# Autodesk Inventor assembly: Ellbow n24_v2
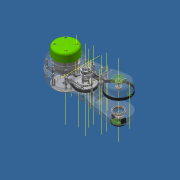
[picture p0: Inventor's stored thumbnail of the model, 180x180]
Saved by Autodesk Inventor 2016 (Build 200138000, 138)
## iProperties
Created: 2015-08-24
Part Number: Ellbow n24_v2
Material: Generisch
Document SubType Name: Assembly
Designer: 4ndreas
Mass: 4151.42 g
Surface Area: 5104.54 cm^2
Volume: 2390.65 cm^3
Density: 1.73652 g/cm^3
Author: 4ndreas
## Documents named in this file (32)
- C:\Users\4ndreas\Documents\Inventor\RobotARM v2\v4\Ellbow n24_v2.iam
- C:\Users\4ndreas\Documents\Inventor\RobotARM v2\v4\Ellbow\Konstruktions-Assistent\Übertragung des Zahnriemens1.iam
- C:\Users\4ndreas\Documents\Inventor\RobotARM v2\v4\Nema24.ipt
- C:\Users\4ndreas\Documents\Inventor\RobotARM v2\v4\Ellbow\Konstruktions-Assistent\Übertragung des Zahnriemens2.iam
- C:\Users\4ndreas\Documents\Inventor\RobotARM v2\v4\OberArm_A.ipt
- C:\Users\4ndreas\Documents\Inventor\RobotARM v2\v4\OberArm_B.ipt
- C:\Users\4ndreas\Documents\Inventor\RobotARM v2\v4\OberArm_C.ipt
- C:\Users\4ndreas\Documents\Inventor\RobotARM v2\v4\Ellbow n24_v2\Konstruktions-Assistent\Welle1.iam
- C:\Users\4ndreas\Documents\Inventor\Content Center Files\R2014\de-DE\DIN BEARING(1)\DIN 625 SKF - SKF 608.ipt
- C:\Users\4ndreas\Documents\Inventor\RobotARM v2\v2\encoder.iam
- C:\Users\4ndreas\Documents\Inventor\RobotARM v2\v4\DIN 912 - M4 x 0,7.ipt
- C:\Users\4ndreas\Documents\Inventor\RobotARM v2\v4\MotorCoverN24_3.ipt
- C:\Users\4ndreas\Documents\Inventor\RobotARM v2\v4\Cover_G2.ipt
- C:\Users\4ndreas\Documents\Inventor\Content Center Files\R2014\de-DE\DIN 912\DIN 912 - M3 x 0,5 x 10 x 8,75.ipt
- C:\Users\4ndreas\Documents\Inventor\Content Center Files\R2014\de-DE\DIN 912\DIN 912 - M4 x 0,7 x 35 x 20.ipt
- C:\Users\4ndreas\Documents\Inventor\Content Center Files\R2014\de-DE\DIN 912\DIN 912 - M4 x 0,7 x 40 x 20.ipt
- C:\Users\4ndreas\Documents\Inventor\Content Center Files\R2014\de-DE\DIN 9021\DIN 9021 - 4,3.ipt
- C:\Users\4ndreas\Documents\Inventor\Content Center Files\R2014\de-DE\DIN 625 - T1\DIN 625 T1 - 624 - 4 x 13 x 5.ipt
- C:\Users\4ndreas\Documents\Inventor\Content Center Files\R2014\de-DE\DIN 125-1  A\DIN 125 - A 4,3.ipt
- C:\Users\4ndreas\Documents\Inventor\RobotARM v2\Diszanzbolzen_M4x20.ipt
- C:\Users\4ndreas\Documents\Inventor\Content Center Files\R2014\de-DE\DIN BEARING(1)\DIN 625 SKF - SKF 61807.ipt
- C:\Users\4ndreas\Documents\Inventor\RobotARM v2\v4\DIN 912 - M4 x 0,7 x55.ipt
- C:\Users\4ndreas\Documents\Inventor\RobotARM v2\v4\16221600.ipt
- C:\Users\4ndreas\Documents\Inventor\RobotARM v2\v4\16224800.ipt
- C:\Users\4ndreas\Documents\Inventor\Content Center Files\R2014\de-DE\DIN 912\DIN 912 - M4 x 0,7 x 30 x 20.ipt
- C:\Users\4ndreas\Documents\Inventor\Content Center Files\R2014\de-DE\DIN 933\DIN 933 - M4  x 55.ipt
- C:\Users\4ndreas\Documents\Inventor\Content Center Files\R2014\de-DE\DIN 934\DIN 934 - M4 x 0,7.ipt
- C:\Users\4ndreas\Documents\Inventor\Content Center Files\R2014\de-DE\DIN 562\DIN 562 - M4 x 7.ipt
- C:\Users\4ndreas\Documents\Inventor\Content Center Files\R2014\de-DE\DIN 933\DIN 933 - M4  x 25.ipt
- C:\Users\4ndreas\Documents\Inventor\RobotARM v2\v4\OberArmMagnet.ipt
- C:\Users\4ndreas\Documents\Inventor\Content Center Files\R2014\de-DE\DIN 7991(2)\DIN 7991 - M4x30.ipt
- C:\Users\4ndreas\Documents\Inventor\Content Center Files\R2014\de-DE\DIN 985\DIN 985 - M4.ipt
## Components (142 placed, 30 different names)
1. Übertragung des Zahnriemens:1 [sub-assembly] — Passend:25, Passend:31, Passend:37, Passend:41, Passend:104, Passend:105, Passend:120, Passend:193
2. Nema24:1 — Passend:3, Passend:16, Winkel:1, Winkel:2, Passend:33, Passend:35, Passend:36, Passend:52, Passend:54, Passend:55, Passend:154, Passend:155, Fluchtend:11
3. Übertragung des Zahnriemens:2 [sub-assembly] — Passend:16, Passend:24, Passend:34, Passend:156
4. OberArm_A:1 — Passend:29, Fluchtend:1, Passend:30, Fluchtend:3, Passend:32, Passend:33, Passend:34, Passend:44, Passend:45, Passend:72, Passend:73, Passend:74, Passend:75, Passend:76, Passend:78, Passend:245, Passend:246, Passend:247, Passend:248, Passend:249
5. OberArm_B:1 — Passend:28, Passend:29, Fluchtend:1, Passend:30, Fluchtend:4, Passend:43, Passend:50, Passend:226, Passend:227, Passend:228, Passend:229, Passend:241, Passend:242, Passend:243, Passend:244, Fluchtend:12
6. OberArm_C:1 — Passend:28, Fluchtend:3, Passend:31, Fluchtend:4, Passend:48, Passend:49, Passend:51, Fluchtend:9, Passend:100, Passend:101, Passend:102, Passend:103, Passend:107, Passend:108, Passend:130, Passend:131, Passend:132, Passend:133, Passend:134, Passend:135, Passend:136, Passend:137, Passend:138, Passend:144, Passend:150, Passend:151, Passend:161, Passend:162, Passend:201, Passend:202, Passend:203, Passend:204, Passend:205, Passend:211, Passend:220, Passend:222, Passend:223, Passend:250, Passend:251, Passend:252, Passend:256
7. Cover_G2:1 — Fluchtend:9, Passend:80, Passend:81, Passend:82, Passend:83, Passend:84, Passend:85, Passend:86, Passend:87
8. Welle:1 [sub-assembly] — Passend:37, Passend:38, Passend:40, Passend:39, Passend:206
9. encoder:1 [sub-assembly] — Passend:41, Passend:43, Passend:256
10. OberArmMagnet:1 — Fluchtend:12, Passend:261, Passend:262, Fluchtend:13, Passend:263, Passend:264, Fluchtend:14, Fluchtend:15
11. DIN 625 SKF SKF 608:1 — Passend:38, Passend:204
12. DIN 625 SKF SKF 608:2 — Passend:39, Passend:205, Passend:207
13. DIN 625 SKF SKF 608:3 — Passend:40, Passend:203
14. DIN 625 SKF SKF 608:4 — Passend:45, Passend:49
15. DIN 625 SKF SKF 608:5 — Passend:50, Passend:51
16. DIN 625 SKF SKF 608:6 — Passend:44, Passend:48
17. DIN 912 - ersetzt durch DIN EN ISO 4762 M4 x 50:5 — Passend:55, Passend:71, Passend:258
18. DIN 912 - ersetzt durch DIN EN ISO 4762 M4 x 50:6 — Passend:54, Passend:69
19. DIN 912 - ersetzt durch DIN EN ISO 4762 M4 x 50:7 — Passend:53, Passend:70
20. DIN 912 - ersetzt durch DIN EN ISO 4762 M4 x 50:8 — Passend:52, Passend:68
21. DIN 125-1 A A 4,3:6
22. DIN 125-1 A A 4,3:7
23. DIN 125-1 A A 4,3:8
24. DIN 125-1 A A 4,3:9
25. Diszanzbolzen_M4x20:5 — Passend:71, Fluchtend:6, Fluchtend:7, Passend:72
26. Diszanzbolzen_M4x20:6 — Passend:69, Fluchtend:6, Passend:73, Passend:88
27. Diszanzbolzen_M4x20:7 — Passend:70, Fluchtend:7, Fluchtend:8, Passend:75, Passend:76
28. Diszanzbolzen_M4x20:8 — Passend:68, Fluchtend:8, Passend:74, Passend:259
29. MotorCoverN24_3:1 — Passend:78, Passend:89, Passend:92, Passend:93, Passend:94, Passend:257, Passend:260
30. DIN 912 - ersetzt durch DIN EN ISO 4762 M3 x 10:1 — Passend:82, Passend:87
31. DIN 912 - ersetzt durch DIN EN ISO 4762 M3 x 10:2 — Passend:81, Passend:86
32. DIN 912 - ersetzt durch DIN EN ISO 4762 M3 x 10:3 — Passend:83, Passend:84
33. DIN 912 - ersetzt durch DIN EN ISO 4762 M3 x 10:4 — Passend:80, Passend:85
34. DIN 912 - ersetzt durch DIN EN ISO 4762 M4 x 35:1 — Passend:88, Passend:89
35. DIN 912 - ersetzt durch DIN EN ISO 4762 M4 x 35:2 — Passend:92, Passend:93, Passend:258
36. DIN 912 - ersetzt durch DIN EN ISO 4762 M4 x 35:3 — Passend:259, Passend:260
37. DIN 912 - ersetzt durch DIN EN ISO 4762 M4 x 35:4 — Passend:90, Passend:94, Passend:257
38. DIN 912 - ersetzt durch DIN EN ISO 4762 M4 x 40:10 — Passend:96, Passend:99, Passend:101, Passend:105, Passend:109, Passend:115, Passend:121, Passend:127
39. DIN 912 - ersetzt durch DIN EN ISO 4762 M4 x 40:9 — Passend:97, Passend:98, Passend:100, Passend:104, Passend:106, Passend:114, Passend:126
40. DIN 9021 4,3:1 — Passend:96, Passend:99, Passend:102
41. DIN 9021 4,3:2 — Passend:97, Passend:98, Passend:103
42. DIN 9021 4,3:3 — Passend:108, Passend:109, Passend:122
43. DIN 9021 4,3:4 — Passend:106, Passend:107, Passend:123
44. DIN 625 - T1 624 - 4 x 13 x 5:1 — Passend:110, Passend:112, Passend:124
45. DIN 625 - T1 624 - 4 x 13 x 5:2 — Passend:110, Passend:112, Passend:115, Passend:129
46. DIN 625 - T1 624 - 4 x 13 x 5:3 — Passend:111, Passend:113, Passend:125
47. DIN 625 - T1 624 - 4 x 13 x 5:4 — Passend:111, Passend:113, Passend:114, Passend:128
48. DIN 125-1 A A 4,3:1 — Passend:117, Passend:119, Passend:125
49. DIN 125-1 A A 4,3:2 — Passend:117, Passend:119, Passend:120, Passend:123
50. DIN 125-1 A A 4,3:3 — Passend:116, Passend:118, Passend:124
51. DIN 125-1 A A 4,3:4 — Passend:116, Passend:118, Passend:121, Passend:122
52. DIN 985 - ersetzt durch DIN EN ISO 10511 M4:1 — Passend:126, Passend:128
53. DIN 985 - ersetzt durch DIN EN ISO 10511 M4:2 — Passend:127, Passend:129
54. DIN 625 SKF SKF 61807:1 — Passend:130, Passend:131
55. Diszanzbolzen_M4x20:9 — Passend:132, Passend:136, Passend:137
56. Diszanzbolzen_M4x20:10 — Passend:133, Passend:134, Passend:135
57. DIN 912 - ersetzt durch DIN EN ISO 4762 M4 x 55:12 — Passend:138
58. DIN 125-1 A A 4,3:10
59. DIN 912 - ersetzt durch DIN EN ISO 4762 M4 x 55:13 — Passend:144
60. DIN 125-1 A A 4,3:11
61. DIN 912 - ersetzt durch DIN EN ISO 4762 M4 x 55:14 — Passend:151
62. DIN 125-1 A A 4,3:12
63. DIN 912 - ersetzt durch DIN EN ISO 4762 M4 x 55:15 — Passend:150
64. DIN 125-1 A A 4,3:13
65. 16221600:1 — Passend:154, Passend:155, Fluchtend:10
66. 16224800:1 — Passend:156, Fluchtend:10
67. DIN 912 - ersetzt durch DIN EN ISO 4762 M4 x 55:16 — Passend:162, Passend:190
68. DIN 912 - ersetzt durch DIN EN ISO 4762 M4 x 55:17 — Passend:161, Passend:165, Passend:188
69. DIN 125-1 A A 4,3:14
70. DIN 125-1 A A 4,3:15
71. DIN 912 - ersetzt durch DIN EN ISO 4762 M4 x 30:1 — Passend:165, Passend:187
72. DIN 125-1 A A 4,3:16
73. DIN 125-1 A A 4,3:17
74. DIN 933 - ersetzt durch DIN EN 24017 M4  x 55:2 — Passend:184, Passend:191, Passend:192, Passend:198
75. DIN 933 - ersetzt durch DIN EN 24017 M4  x 55:1 — Passend:183, Passend:194, Passend:196
76. DIN 125-1 A A 4,3:18
77. DIN 125-1 A A 4,3:19
78. DIN 934 - ersetzt durch DIN EN 24032/28673/28674 M4:1 — Passend:188
79. DIN 934 - ersetzt durch DIN EN 24032/28673/28674 M4:2 — Passend:187
80. DIN 934 - ersetzt durch DIN EN 24032/28673/28674 M4:3 — Passend:184
81. DIN 934 - ersetzt durch DIN EN 24032/28673/28674 M4:4 — Passend:183
82. DIN 934 - ersetzt durch DIN EN 24032/28673/28674 M4:6 — Passend:190
83. DIN 625 - T1 624 - 4 x 13 x 5:5 — Passend:193, Passend:195, Passend:197
84. DIN 625 - T1 624 - 4 x 13 x 5:6 — Passend:192, Passend:199, Passend:201
85. DIN 625 - T1 624 - 4 x 13 x 5:7 — Passend:191, Passend:199, Passend:200
86. DIN 625 - T1 624 - 4 x 13 x 5:8 — Passend:194, Passend:195, Passend:202
87. DIN 934 - ersetzt durch DIN EN 24032/28673/28674 M4:7 — Passend:196, Passend:197
88. DIN 934 - ersetzt durch DIN EN 24032/28673/28674 M4:8 — Passend:198, Passend:200
89. 16221600:2 — Passend:206, Passend:207
90. DIN 912 - ersetzt durch DIN EN ISO 4762 M4 x 55:18 — Passend:211, Passend:239
91. DIN 125-1 A A 4,3:20
92. DIN 912 - ersetzt durch DIN EN ISO 4762 M4 x 55:19 — Passend:220, Passend:240
93. DIN 912 - ersetzt durch DIN EN ISO 4762 M4 x 55:20 — Passend:222, Passend:238
94. DIN 912 - ersetzt durch DIN EN ISO 4762 M4 x 55:21 — Passend:223, Passend:237
95. DIN 125-1 A A 4,3:21
96. DIN 125-1 A A 4,3:5
97. DIN 125-1 A A 4,3:22
98. DIN 562 M4:1 — Passend:239, Passend:245, Passend:246
99. DIN 562 M4:2 — Passend:240, Passend:241, Passend:242
100. DIN 562 M4:3 — Passend:237, Passend:247, Passend:248
101. DIN 562 M4:4 — Passend:238, Passend:243, Passend:244
102. DIN 933 - ersetzt durch DIN EN 24017 M4  x 25:1 — Passend:250, Passend:251, Passend:252, Passend:254
103. DIN 934 - ersetzt durch DIN EN 24032/28673/28674 M4:9 — Passend:254
104. DIN 7991 M4x30:2 — Passend:262, Fluchtend:13
105. DIN 7991 M4x30:3 — Passend:263, Fluchtend:14
106. DIN 7991 M4x30:4 — Passend:264, Fluchtend:15
107. DIN 7991 M4x30:1
108. DIN 912 - ersetzt durch DIN EN ISO 4762 M4 x 30:5 — Passend:229
109. DIN 125-1 A A 4,3:23
110. Diszanzbolzen_M4x20:11 — Passend:226, Passend:227, Passend:228, Passend:235
111. DIN 912 - ersetzt durch DIN EN ISO 4762 M4 x 30:4 — Passend:235
112. DIN 125-1 A A 4,3:24
113. DIN 912 - ersetzt durch DIN EN ISO 4762 M4 x 30:6
114. DIN 125-1 A A 4,3:25
115. Diszanzbolzen_M4x20:12
116. DIN 912 - ersetzt durch DIN EN ISO 4762 M4 x 30:7
117. DIN 125-1 A A 4,3:26
118. DIN 912 - ersetzt durch DIN EN ISO 4762 M4 x 30:8
119. DIN 125-1 A A 4,3:27
120. Diszanzbolzen_M4x20:13
121. DIN 912 - ersetzt durch DIN EN ISO 4762 M4 x 30:9
122. DIN 125-1 A A 4,3:28
123. DIN 912 - ersetzt durch DIN EN ISO 4762 M4 x 30:10
124. DIN 125-1 A A 4,3:29
125. Diszanzbolzen_M4x20:14
126. DIN 912 - ersetzt durch DIN EN ISO 4762 M4 x 30:11
127. DIN 125-1 A A 4,3:30
128. DIN 912 - ersetzt durch DIN EN ISO 4762 M4 x 30:12
129. DIN 125-1 A A 4,3:31
130. Diszanzbolzen_M4x20:15
131. DIN 912 - ersetzt durch DIN EN ISO 4762 M4 x 30:13
132. DIN 125-1 A A 4,3:32
133. DIN 912 - ersetzt durch DIN EN ISO 4762 M4 x 30:14
134. DIN 125-1 A A 4,3:33
135. Diszanzbolzen_M4x20:16
136. DIN 912 - ersetzt durch DIN EN ISO 4762 M4 x 30:15
137. DIN 125-1 A A 4,3:34
138. DIN 912 - ersetzt durch DIN EN ISO 4762 M4 x 30:16
139. DIN 125-1 A A 4,3:35
140. Diszanzbolzen_M4x20:17
141. DIN 912 - ersetzt durch DIN EN ISO 4762 M4 x 30:17
142. DIN 125-1 A A 4,3:36
## Component patterns: (7 elements, first: DIN 912 - ersetzt durch DIN EN ISO 4762 M4 x 30:5 + DIN 125-1 A A 4,3:23 + Diszanzbolzen_M4x20:11 + DIN 912 - ersetzt durch DIN EN ISO 4762 M4 x 30:4 + DIN 125-1 A A 4,3:24)
## Relationships (247: Mate 231, Flush 14, Angle 2)
- Passend:3 [Mate]: Nema24:1
- Passend:12 [Mate]
- Passend:13 [Mate]
- Passend:16 [Mate]: Nema24:1 ↔ Übertragung des Zahnriemens:2
- Winkel:1 [Angle] (0 deg): Nema24:1
- Passend:24 [Mate]: Übertragung des Zahnriemens:2
- Passend:25 [Mate]: Übertragung des Zahnriemens:1
- Winkel:2 [Angle] (180 deg): Nema24:1
- Passend:28 [Mate]: OberArm_B:1 ↔ OberArm_C:1
- Passend:29 [Mate]: OberArm_A:1 ↔ OberArm_B:1
- Fluchtend:1 [Flush]: OberArm_A:1 ↔ OberArm_B:1
- Passend:30 [Mate]: OberArm_A:1 ↔ OberArm_B:1
- Fluchtend:3 [Flush]: OberArm_A:1 ↔ OberArm_C:1
- Passend:31 [Mate]: Übertragung des Zahnriemens:1 ↔ OberArm_C:1
- Passend:32 [Mate]: OberArm_A:1
- Passend:33 [Mate]: Nema24:1 ↔ OberArm_A:1
- Passend:34 [Mate]: Übertragung des Zahnriemens:2 ↔ OberArm_A:1
- Passend:35 [Mate]: Nema24:1
- Passend:36 [Mate]: Nema24:1
- Fluchtend:4 [Flush]: OberArm_B:1 ↔ OberArm_C:1
- Passend:37 [Mate]: Übertragung des Zahnriemens:1 ↔ Welle:1
- Passend:38 [Mate]: Welle:1 ↔ DIN 625 SKF SKF 608:1
- Passend:39 [Mate]: Welle:1 ↔ DIN 625 SKF SKF 608:2
- Passend:40 [Mate]: Welle:1 ↔ DIN 625 SKF SKF 608:3
- Passend:41 [Mate]: Übertragung des Zahnriemens:1 ↔ encoder:1
- Passend:43 [Mate]: OberArm_B:1 ↔ encoder:1
- Passend:44 [Mate]: OberArm_A:1 ↔ DIN 625 SKF SKF 608:6
- Passend:45 [Mate]: OberArm_A:1 ↔ DIN 625 SKF SKF 608:4
- Passend:48 [Mate]: OberArm_C:1 ↔ DIN 625 SKF SKF 608:6
- Passend:49 [Mate]: OberArm_C:1 ↔ DIN 625 SKF SKF 608:4
- Passend:50 [Mate]: OberArm_B:1 ↔ DIN 625 SKF SKF 608:5
- Passend:51 [Mate]: OberArm_C:1 ↔ DIN 625 SKF SKF 608:5
- Passend:52 [Mate]: Nema24:1 ↔ DIN 912 - ersetzt durch DIN EN ISO 4762 M4 x 50:8
- Passend:53 [Mate]: DIN 912 - ersetzt durch DIN EN ISO 4762 M4 x 50:7
- Passend:54 [Mate]: Nema24:1 ↔ DIN 912 - ersetzt durch DIN EN ISO 4762 M4 x 50:6
- Passend:55 [Mate]: Nema24:1 ↔ DIN 912 - ersetzt durch DIN EN ISO 4762 M4 x 50:5
- [Mate]: DIN 912 - ersetzt durch DIN EN ISO 4762 M4 x 50:8 ↔ DIN 125-1 A A 4,3:7
- [Mate]: DIN 912 - ersetzt durch DIN EN ISO 4762 M4 x 50:6 ↔ DIN 125-1 A A 4,3:6
- [Mate]: DIN 912 - ersetzt durch DIN EN ISO 4762 M4 x 50:5 ↔ DIN 125-1 A A 4,3:9
- [Mate]: DIN 912 - ersetzt durch DIN EN ISO 4762 M4 x 50:7 ↔ DIN 125-1 A A 4,3:8
- [Mate]: DIN 912 - ersetzt durch DIN EN ISO 4762 M4 x 50:7 ↔ DIN 125-1 A A 4,3:8
- [Mate]: DIN 912 - ersetzt durch DIN EN ISO 4762 M4 x 50:8 ↔ DIN 125-1 A A 4,3:7
- [Mate]: DIN 912 - ersetzt durch DIN EN ISO 4762 M4 x 50:6 ↔ DIN 125-1 A A 4,3:6
- [Mate]: DIN 912 - ersetzt durch DIN EN ISO 4762 M4 x 50:5 ↔ DIN 125-1 A A 4,3:9
- [Mate]: Nema24:1 ↔ DIN 125-1 A A 4,3:6
- [Mate]: Nema24:1 ↔ DIN 125-1 A A 4,3:7
- [Mate]: Nema24:1 ↔ DIN 125-1 A A 4,3:9
- [Mate]: Nema24:1 ↔ DIN 125-1 A A 4,3:8
- Passend:68 [Mate]: DIN 912 - ersetzt durch DIN EN ISO 4762 M4 x 50:8 ↔ Diszanzbolzen_M4x20:8
- Passend:69 [Mate]: DIN 912 - ersetzt durch DIN EN ISO 4762 M4 x 50:6 ↔ Diszanzbolzen_M4x20:6
- Passend:70 [Mate]: DIN 912 - ersetzt durch DIN EN ISO 4762 M4 x 50:7 ↔ Diszanzbolzen_M4x20:7
- Passend:71 [Mate]: DIN 912 - ersetzt durch DIN EN ISO 4762 M4 x 50:5 ↔ Diszanzbolzen_M4x20:5
- Fluchtend:6 [Flush]: Diszanzbolzen_M4x20:5 ↔ Diszanzbolzen_M4x20:6
- Fluchtend:7 [Flush]: Diszanzbolzen_M4x20:5 ↔ Diszanzbolzen_M4x20:7
- Fluchtend:8 [Flush]: Diszanzbolzen_M4x20:7 ↔ Diszanzbolzen_M4x20:8
- Passend:72 [Mate]: OberArm_A:1 ↔ Diszanzbolzen_M4x20:5
- Passend:73 [Mate]: OberArm_A:1 ↔ Diszanzbolzen_M4x20:6
- Passend:74 [Mate]: OberArm_A:1 ↔ Diszanzbolzen_M4x20:8
- Passend:75 [Mate]: OberArm_A:1 ↔ Diszanzbolzen_M4x20:7
- Passend:76 [Mate]: OberArm_A:1 ↔ Diszanzbolzen_M4x20:7
- Passend:78 [Mate]: OberArm_A:1 ↔ MotorCoverN24_3:1
- Fluchtend:9 [Flush]: OberArm_C:1 ↔ Cover_G2:1
- Passend:80 [Mate]: Cover_G2:1 ↔ DIN 912 - ersetzt durch DIN EN ISO 4762 M3 x 10:4
- Passend:81 [Mate]: Cover_G2:1 ↔ DIN 912 - ersetzt durch DIN EN ISO 4762 M3 x 10:2
- Passend:82 [Mate]: Cover_G2:1 ↔ DIN 912 - ersetzt durch DIN EN ISO 4762 M3 x 10:1
- Passend:83 [Mate]: Cover_G2:1 ↔ DIN 912 - ersetzt durch DIN EN ISO 4762 M3 x 10:3
- Passend:84 [Mate]: Cover_G2:1 ↔ DIN 912 - ersetzt durch DIN EN ISO 4762 M3 x 10:3
- Passend:85 [Mate]: Cover_G2:1 ↔ DIN 912 - ersetzt durch DIN EN ISO 4762 M3 x 10:4
- Passend:86 [Mate]: Cover_G2:1 ↔ DIN 912 - ersetzt durch DIN EN ISO 4762 M3 x 10:2
- Passend:87 [Mate]: Cover_G2:1 ↔ DIN 912 - ersetzt durch DIN EN ISO 4762 M3 x 10:1
- Passend:88 [Mate]: Diszanzbolzen_M4x20:6 ↔ DIN 912 - ersetzt durch DIN EN ISO 4762 M4 x 35:1
- Passend:89 [Mate]: MotorCoverN24_3:1 ↔ DIN 912 - ersetzt durch DIN EN ISO 4762 M4 x 35:1
- Passend:90 [Mate]: DIN 912 - ersetzt durch DIN EN ISO 4762 M4 x 35:4
- Passend:92 [Mate]: MotorCoverN24_3:1 ↔ DIN 912 - ersetzt durch DIN EN ISO 4762 M4 x 35:2
- Passend:93 [Mate]: MotorCoverN24_3:1 ↔ DIN 912 - ersetzt durch DIN EN ISO 4762 M4 x 35:2
- Passend:94 [Mate]: MotorCoverN24_3:1 ↔ DIN 912 - ersetzt durch DIN EN ISO 4762 M4 x 35:4
- Passend:96 [Mate]: DIN 912 - ersetzt durch DIN EN ISO 4762 M4 x 40:10 ↔ DIN 9021 4,3:1
- Passend:97 [Mate]: DIN 912 - ersetzt durch DIN EN ISO 4762 M4 x 40:9 ↔ DIN 9021 4,3:2
- Passend:98 [Mate]: DIN 912 - ersetzt durch DIN EN ISO 4762 M4 x 40:9 ↔ DIN 9021 4,3:2
- Passend:99 [Mate]: DIN 912 - ersetzt durch DIN EN ISO 4762 M4 x 40:10 ↔ DIN 9021 4,3:1
- Passend:100 [Mate]: OberArm_C:1 ↔ DIN 912 - ersetzt durch DIN EN ISO 4762 M4 x 40:9
- Passend:101 [Mate]: OberArm_C:1 ↔ DIN 912 - ersetzt durch DIN EN ISO 4762 M4 x 40:10
- Passend:102 [Mate]: OberArm_C:1 ↔ DIN 9021 4,3:1
- Passend:103 [Mate]: OberArm_C:1 ↔ DIN 9021 4,3:2
- Passend:104 [Mate]: Übertragung des Zahnriemens:1 ↔ DIN 912 - ersetzt durch DIN EN ISO 4762 M4 x 40:9
- Passend:105 [Mate]: Übertragung des Zahnriemens:1 ↔ DIN 912 - ersetzt durch DIN EN ISO 4762 M4 x 40:10
- Passend:106 [Mate]: DIN 912 - ersetzt durch DIN EN ISO 4762 M4 x 40:9 ↔ DIN 9021 4,3:4
- Passend:107 [Mate]: OberArm_C:1 ↔ DIN 9021 4,3:4
- Passend:108 [Mate]: OberArm_C:1 ↔ DIN 9021 4,3:3
- Passend:109 [Mate]: DIN 912 - ersetzt durch DIN EN ISO 4762 M4 x 40:10 ↔ DIN 9021 4,3:3
- Passend:110 [Mate]: DIN 625 - T1 624 - 4 x 13 x 5:1 ↔ DIN 625 - T1 624 - 4 x 13 x 5:2
- Passend:111 [Mate]: DIN 625 - T1 624 - 4 x 13 x 5:3 ↔ DIN 625 - T1 624 - 4 x 13 x 5:4
- Passend:112 [Mate]: DIN 625 - T1 624 - 4 x 13 x 5:1 ↔ DIN 625 - T1 624 - 4 x 13 x 5:2
- Passend:113 [Mate]: DIN 625 - T1 624 - 4 x 13 x 5:3 ↔ DIN 625 - T1 624 - 4 x 13 x 5:4
- Passend:114 [Mate]: DIN 912 - ersetzt durch DIN EN ISO 4762 M4 x 40:9 ↔ DIN 625 - T1 624 - 4 x 13 x 5:4
- Passend:115 [Mate]: DIN 912 - ersetzt durch DIN EN ISO 4762 M4 x 40:10 ↔ DIN 625 - T1 624 - 4 x 13 x 5:2
- Passend:116 [Mate]: DIN 125-1 A A 4,3:3 ↔ DIN 125-1 A A 4,3:4
- Passend:117 [Mate]: DIN 125-1 A A 4,3:1 ↔ DIN 125-1 A A 4,3:2
- Passend:118 [Mate]: DIN 125-1 A A 4,3:3 ↔ DIN 125-1 A A 4,3:4
- Passend:119 [Mate]: DIN 125-1 A A 4,3:1 ↔ DIN 125-1 A A 4,3:2
- Passend:120 [Mate]: Übertragung des Zahnriemens:1 ↔ DIN 125-1 A A 4,3:2
- Passend:121 [Mate]: DIN 912 - ersetzt durch DIN EN ISO 4762 M4 x 40:10 ↔ DIN 125-1 A A 4,3:4
- Passend:122 [Mate]: DIN 9021 4,3:3 ↔ DIN 125-1 A A 4,3:4
- Passend:123 [Mate]: DIN 9021 4,3:4 ↔ DIN 125-1 A A 4,3:2
- Passend:124 [Mate]: DIN 625 - T1 624 - 4 x 13 x 5:1 ↔ DIN 125-1 A A 4,3:3
- Passend:125 [Mate]: DIN 625 - T1 624 - 4 x 13 x 5:3 ↔ DIN 125-1 A A 4,3:1
- Passend:126 [Mate]: DIN 912 - ersetzt durch DIN EN ISO 4762 M4 x 40:9 ↔ DIN 985 - ersetzt durch DIN EN ISO 10511 M4:1
- Passend:127 [Mate]: DIN 912 - ersetzt durch DIN EN ISO 4762 M4 x 40:10 ↔ DIN 985 - ersetzt durch DIN EN ISO 10511 M4:2
- Passend:128 [Mate]: DIN 625 - T1 624 - 4 x 13 x 5:4 ↔ DIN 985 - ersetzt durch DIN EN ISO 10511 M4:1
- Passend:129 [Mate]: DIN 625 - T1 624 - 4 x 13 x 5:2 ↔ DIN 985 - ersetzt durch DIN EN ISO 10511 M4:2
- Passend:130 [Mate]: OberArm_C:1 ↔ DIN 625 SKF SKF 61807:1
- Passend:131 [Mate]: OberArm_C:1 ↔ DIN 625 SKF SKF 61807:1
- Passend:132 [Mate]: OberArm_C:1 ↔ Diszanzbolzen_M4x20:9
- Passend:133 [Mate]: OberArm_C:1 ↔ Diszanzbolzen_M4x20:10
- Passend:134 [Mate]: OberArm_C:1 ↔ Diszanzbolzen_M4x20:10
- Passend:135 [Mate]: OberArm_C:1 ↔ Diszanzbolzen_M4x20:10
- Passend:136 [Mate]: OberArm_C:1 ↔ Diszanzbolzen_M4x20:9
- Passend:137 [Mate]: OberArm_C:1 ↔ Diszanzbolzen_M4x20:9
- Passend:138 [Mate]: OberArm_C:1 ↔ DIN 912 - ersetzt durch DIN EN ISO 4762 M4 x 55:12
- [Mate]: DIN 912 - ersetzt durch DIN EN ISO 4762 M4 x 55:12 ↔ DIN 125-1 A A 4,3:10
- [Mate]: DIN 912 - ersetzt durch DIN EN ISO 4762 M4 x 55:12 ↔ DIN 125-1 A A 4,3:10
- [Mate]: OberArm_C:1 ↔ DIN 125-1 A A 4,3:10
- [Mate]: DIN 912 - ersetzt durch DIN EN ISO 4762 M4 x 55:13 ↔ DIN 125-1 A A 4,3:11
- [Mate]: DIN 912 - ersetzt durch DIN EN ISO 4762 M4 x 55:13 ↔ DIN 125-1 A A 4,3:11
- Passend:144 [Mate]: OberArm_C:1 ↔ DIN 912 - ersetzt durch DIN EN ISO 4762 M4 x 55:13
- [Mate]: OberArm_C:1 ↔ DIN 125-1 A A 4,3:11
- [Mate]: DIN 912 - ersetzt durch DIN EN ISO 4762 M4 x 55:14 ↔ DIN 125-1 A A 4,3:12
- [Mate]: DIN 912 - ersetzt durch DIN EN ISO 4762 M4 x 55:14 ↔ DIN 125-1 A A 4,3:12
- [Mate]: DIN 912 - ersetzt durch DIN EN ISO 4762 M4 x 55:15 ↔ DIN 125-1 A A 4,3:13
- [Mate]: DIN 912 - ersetzt durch DIN EN ISO 4762 M4 x 55:15 ↔ DIN 125-1 A A 4,3:13
- Passend:150 [Mate]: OberArm_C:1 ↔ DIN 912 - ersetzt durch DIN EN ISO 4762 M4 x 55:15
- Passend:151 [Mate]: OberArm_C:1 ↔ DIN 912 - ersetzt durch DIN EN ISO 4762 M4 x 55:14
- [Mate]: OberArm_C:1 ↔ DIN 125-1 A A 4,3:12
- [Mate]: OberArm_C:1 ↔ DIN 125-1 A A 4,3:13
- Passend:154 [Mate]: Nema24:1 ↔ 16221600:1
- Passend:155 [Mate] (1 mm): Nema24:1 ↔ 16221600:1
- Passend:156 [Mate]: Übertragung des Zahnriemens:2 ↔ 16224800:1
- Fluchtend:10 [Flush]: 16221600:1 ↔ 16224800:1
- Fluchtend:11 [Flush] (7 mm): Nema24:1
- [Mate]: DIN 912 - ersetzt durch DIN EN ISO 4762 M4 x 55:17 ↔ DIN 125-1 A A 4,3:15
- [Mate]: DIN 912 - ersetzt durch DIN EN ISO 4762 M4 x 55:16 ↔ DIN 125-1 A A 4,3:14
- [Mate]: DIN 912 - ersetzt durch DIN EN ISO 4762 M4 x 55:16 ↔ DIN 125-1 A A 4,3:14
- [Mate]: DIN 912 - ersetzt durch DIN EN ISO 4762 M4 x 55:17 ↔ DIN 125-1 A A 4,3:15
- Passend:161 [Mate]: OberArm_C:1 ↔ DIN 912 - ersetzt durch DIN EN ISO 4762 M4 x 55:17
- Passend:162 [Mate]: OberArm_C:1 ↔ DIN 912 - ersetzt durch DIN EN ISO 4762 M4 x 55:16
- [Mate]: OberArm_C:1 ↔ DIN 125-1 A A 4,3:14
- [Mate]: OberArm_C:1 ↔ DIN 125-1 A A 4,3:15
- Passend:165 [Mate]: DIN 912 - ersetzt durch DIN EN ISO 4762 M4 x 55:17 ↔ DIN 912 - ersetzt durch DIN EN ISO 4762 M4 x 30:1
- [Mate]: DIN 912 - ersetzt durch DIN EN ISO 4762 M4 x 30:1 ↔ DIN 125-1 A A 4,3:17
- [Mate]: DIN 912 - ersetzt durch DIN EN ISO 4762 M4 x 30:1 ↔ DIN 125-1 A A 4,3:17
- [Mate]: OberArm_C:1 ↔ DIN 125-1 A A 4,3:16
- [Mate]: OberArm_C:1 ↔ DIN 125-1 A A 4,3:17
- [Mate]: Übertragung des Zahnriemens:1 ↔ DIN 933 - ersetzt durch DIN EN 24017 M4  x 55:2
- [Mate]: Übertragung des Zahnriemens:1 ↔ DIN 933 - ersetzt durch DIN EN 24017 M4  x 55:1
- [Mate]: OberArm_C:1 ↔ DIN 933 - ersetzt durch DIN EN 24017 M4  x 55:2
- [Mate]: OberArm_C:1 ↔ DIN 933 - ersetzt durch DIN EN 24017 M4  x 55:1
- [Mate]: OberArm_C:1 ↔ DIN 933 - ersetzt durch DIN EN 24017 M4  x 55:2
- [Mate]: OberArm_C:1 ↔ DIN 933 - ersetzt durch DIN EN 24017 M4  x 55:1
- [Mate]: OberArm_C:1 ↔ DIN 125-1 A A 4,3:18
- [Mate]: OberArm_C:1 ↔ DIN 125-1 A A 4,3:19
- [Mate]: DIN 933 - ersetzt durch DIN EN 24017 M4  x 55:2 ↔ DIN 125-1 A A 4,3:19
- [Mate]: DIN 933 - ersetzt durch DIN EN 24017 M4  x 55:1 ↔ DIN 125-1 A A 4,3:18
- Passend:183 [Mate]: DIN 933 - ersetzt durch DIN EN 24017 M4  x 55:1 ↔ DIN 934 - ersetzt durch DIN EN 24032/28673/28674 M4:4
- Passend:184 [Mate]: DIN 933 - ersetzt durch DIN EN 24017 M4  x 55:2 ↔ DIN 934 - ersetzt durch DIN EN 24032/28673/28674 M4:3
- [Mate]: DIN 125-1 A A 4,3:19 ↔ DIN 934 - ersetzt durch DIN EN 24032/28673/28674 M4:3
- [Mate]: DIN 125-1 A A 4,3:18 ↔ DIN 934 - ersetzt durch DIN EN 24032/28673/28674 M4:4
- Passend:187 [Mate]: DIN 912 - ersetzt durch DIN EN ISO 4762 M4 x 30:1 ↔ DIN 934 - ersetzt durch DIN EN 24032/28673/28674 M4:2
- Passend:188 [Mate]: DIN 912 - ersetzt durch DIN EN ISO 4762 M4 x 55:17 ↔ DIN 934 - ersetzt durch DIN EN 24032/28673/28674 M4:1
- Passend:190 [Mate]: DIN 912 - ersetzt durch DIN EN ISO 4762 M4 x 55:16 ↔ DIN 934 - ersetzt durch DIN EN 24032/28673/28674 M4:6
- Passend:191 [Mate]: DIN 933 - ersetzt durch DIN EN 24017 M4  x 55:2 ↔ DIN 625 - T1 624 - 4 x 13 x 5:7
- Passend:192 [Mate]: DIN 933 - ersetzt durch DIN EN 24017 M4  x 55:2 ↔ DIN 625 - T1 624 - 4 x 13 x 5:6
- Passend:193 [Mate]: Übertragung des Zahnriemens:1 ↔ DIN 625 - T1 624 - 4 x 13 x 5:5
- Passend:194 [Mate]: DIN 933 - ersetzt durch DIN EN 24017 M4  x 55:1 ↔ DIN 625 - T1 624 - 4 x 13 x 5:8
- Passend:195 [Mate]: DIN 625 - T1 624 - 4 x 13 x 5:5 ↔ DIN 625 - T1 624 - 4 x 13 x 5:8
- Passend:196 [Mate]: DIN 933 - ersetzt durch DIN EN 24017 M4  x 55:1 ↔ DIN 934 - ersetzt durch DIN EN 24032/28673/28674 M4:7
- Passend:197 [Mate]: DIN 625 - T1 624 - 4 x 13 x 5:5 ↔ DIN 934 - ersetzt durch DIN EN 24032/28673/28674 M4:7
- Passend:198 [Mate]: DIN 933 - ersetzt durch DIN EN 24017 M4  x 55:2 ↔ DIN 934 - ersetzt durch DIN EN 24032/28673/28674 M4:8
- Passend:199 [Mate]: DIN 625 - T1 624 - 4 x 13 x 5:6 ↔ DIN 625 - T1 624 - 4 x 13 x 5:7
- Passend:200 [Mate]: DIN 625 - T1 624 - 4 x 13 x 5:7 ↔ DIN 934 - ersetzt durch DIN EN 24032/28673/28674 M4:8
- Passend:201 [Mate]: OberArm_C:1 ↔ DIN 625 - T1 624 - 4 x 13 x 5:6
- Passend:202 [Mate]: OberArm_C:1 ↔ DIN 625 - T1 624 - 4 x 13 x 5:8
- Passend:203 [Mate]: OberArm_C:1 ↔ DIN 625 SKF SKF 608:3
- Passend:204 [Mate]: OberArm_C:1 ↔ DIN 625 SKF SKF 608:1
- Passend:205 [Mate]: OberArm_C:1 ↔ DIN 625 SKF SKF 608:2
- Passend:206 [Mate]: Welle:1 ↔ 16221600:2
- Passend:207 [Mate] (0.5 mm): DIN 625 SKF SKF 608:2 ↔ 16221600:2
- [Mate]: DIN 912 - ersetzt durch DIN EN ISO 4762 M4 x 55:18 ↔ DIN 125-1 A A 4,3:20
- [Mate]: DIN 912 - ersetzt durch DIN EN ISO 4762 M4 x 55:18 ↔ DIN 125-1 A A 4,3:20
- [Mate]: OberArm_C:1 ↔ DIN 125-1 A A 4,3:20
- Passend:211 [Mate]: OberArm_C:1 ↔ DIN 912 - ersetzt durch DIN EN ISO 4762 M4 x 55:18
- [Mate]: DIN 912 - ersetzt durch DIN EN ISO 4762 M4 x 55:19 ↔ DIN 125-1 A A 4,3:21
- [Mate]: DIN 912 - ersetzt durch DIN EN ISO 4762 M4 x 55:20 ↔ DIN 125-1 A A 4,3:22
- [Mate]: DIN 912 - ersetzt durch DIN EN ISO 4762 M4 x 55:21 ↔ DIN 125-1 A A 4,3:5
- [Mate]: DIN 912 - ersetzt durch DIN EN ISO 4762 M4 x 55:20 ↔ DIN 125-1 A A 4,3:22
- [Mate]: DIN 912 - ersetzt durch DIN EN ISO 4762 M4 x 55:19 ↔ DIN 125-1 A A 4,3:21
- [Mate]: DIN 912 - ersetzt durch DIN EN ISO 4762 M4 x 55:21 ↔ DIN 125-1 A A 4,3:5
- Passend:220 [Mate]: OberArm_C:1 ↔ DIN 912 - ersetzt durch DIN EN ISO 4762 M4 x 55:19
- [Mate]: OberArm_C:1 ↔ DIN 125-1 A A 4,3:21
- Passend:222 [Mate]: OberArm_C:1 ↔ DIN 912 - ersetzt durch DIN EN ISO 4762 M4 x 55:20
- Passend:223 [Mate]: OberArm_C:1 ↔ DIN 912 - ersetzt durch DIN EN ISO 4762 M4 x 55:21
- [Mate]: OberArm_C:1 ↔ DIN 125-1 A A 4,3:5
- [Mate]: OberArm_C:1 ↔ DIN 125-1 A A 4,3:22
- Passend:226 [Mate]: OberArm_B:1 ↔ Diszanzbolzen_M4x20:11
- Passend:227 [Mate]: OberArm_B:1 ↔ Diszanzbolzen_M4x20:11
- Passend:228 [Mate]: OberArm_B:1 ↔ Diszanzbolzen_M4x20:11
- Passend:229 [Mate]: OberArm_B:1 ↔ DIN 912 - ersetzt durch DIN EN ISO 4762 M4 x 30:5
- [Mate]: DIN 912 - ersetzt durch DIN EN ISO 4762 M4 x 30:5 ↔ DIN 125-1 A A 4,3:23
- [Mate]: DIN 912 - ersetzt durch DIN EN ISO 4762 M4 x 30:5 ↔ DIN 125-1 A A 4,3:23
- [Mate]: OberArm_B:1 ↔ DIN 125-1 A A 4,3:23
- [Mate]: DIN 912 - ersetzt durch DIN EN ISO 4762 M4 x 30:4 ↔ DIN 125-1 A A 4,3:24
- [Mate]: DIN 912 - ersetzt durch DIN EN ISO 4762 M4 x 30:4 ↔ DIN 125-1 A A 4,3:24
- Passend:235 [Mate]: Diszanzbolzen_M4x20:11 ↔ DIN 912 - ersetzt durch DIN EN ISO 4762 M4 x 30:4
- [Mate]: OberArm_A:1 ↔ DIN 125-1 A A 4,3:24
- Passend:237 [Mate]: DIN 912 - ersetzt durch DIN EN ISO 4762 M4 x 55:21 ↔ DIN 562 M4:3
- Passend:238 [Mate]: DIN 912 - ersetzt durch DIN EN ISO 4762 M4 x 55:20 ↔ DIN 562 M4:4
- Passend:239 [Mate]: DIN 912 - ersetzt durch DIN EN ISO 4762 M4 x 55:18 ↔ DIN 562 M4:1
- Passend:240 [Mate]: DIN 912 - ersetzt durch DIN EN ISO 4762 M4 x 55:19 ↔ DIN 562 M4:2
- Passend:241 [Mate]: OberArm_B:1 ↔ DIN 562 M4:2
- Passend:242 [Mate]: OberArm_B:1 ↔ DIN 562 M4:2
- Passend:243 [Mate]: OberArm_B:1 ↔ DIN 562 M4:4
- Passend:244 [Mate]: OberArm_B:1 ↔ DIN 562 M4:4
- Passend:245 [Mate]: OberArm_A:1 ↔ DIN 562 M4:1
- Passend:246 [Mate]: OberArm_A:1 ↔ DIN 562 M4:1
- Passend:247 [Mate]: OberArm_A:1 ↔ DIN 562 M4:3
- Passend:248 [Mate]: OberArm_A:1 ↔ DIN 562 M4:3
- Passend:249 [Mate]: OberArm_A:1
- Passend:250 [Mate]: OberArm_C:1 ↔ DIN 933 - ersetzt durch DIN EN 24017 M4  x 25:1
- Passend:251 [Mate]: OberArm_C:1 ↔ DIN 933 - ersetzt durch DIN EN 24017 M4  x 25:1
- Passend:252 [Mate]: OberArm_C:1 ↔ DIN 933 - ersetzt durch DIN EN 24017 M4  x 25:1
- [Mate]: DIN 125-1 A A 4,3:16 ↔ DIN 933 - ersetzt durch DIN EN 24017 M4  x 25:1
- Passend:254 [Mate]: DIN 933 - ersetzt durch DIN EN 24017 M4  x 25:1 ↔ DIN 934 - ersetzt durch DIN EN 24032/28673/28674 M4:9
- [Mate]: DIN 125-1 A A 4,3:16 ↔ DIN 934 - ersetzt durch DIN EN 24032/28673/28674 M4:9
- Passend:256 [Mate]: OberArm_C:1 ↔ encoder:1
- Passend:257 [Mate]: MotorCoverN24_3:1 ↔ DIN 912 - ersetzt durch DIN EN ISO 4762 M4 x 35:4
- Passend:258 [Mate]: DIN 912 - ersetzt durch DIN EN ISO 4762 M4 x 50:5 ↔ DIN 912 - ersetzt durch DIN EN ISO 4762 M4 x 35:2
- Passend:259 [Mate]: Diszanzbolzen_M4x20:8 ↔ DIN 912 - ersetzt durch DIN EN ISO 4762 M4 x 35:3
- Passend:260 [Mate]: MotorCoverN24_3:1 ↔ DIN 912 - ersetzt durch DIN EN ISO 4762 M4 x 35:3
- Fluchtend:12 [Flush]: OberArm_B:1 ↔ OberArmMagnet:1
- Passend:261 [Mate]: OberArmMagnet:1
- Passend:262 [Mate]: OberArmMagnet:1 ↔ DIN 7991 M4x30:2
- Fluchtend:13 [Flush]: OberArmMagnet:1 ↔ DIN 7991 M4x30:2
- Passend:263 [Mate]: OberArmMagnet:1 ↔ DIN 7991 M4x30:3
- Passend:264 [Mate]: OberArmMagnet:1 ↔ DIN 7991 M4x30:4
- Fluchtend:14 [Flush]: OberArmMagnet:1 ↔ DIN 7991 M4x30:3
- Fluchtend:15 [Flush]: OberArmMagnet:1 ↔ DIN 7991 M4x30:4
- [Mate]: OberArmMagnet:1 ↔ DIN 7991 M4x30:1
- [Flush]: OberArmMagnet:1 ↔ DIN 7991 M4x30:1
